# Autodesk Inventor assembly: Subensamble_cortadora_MIR
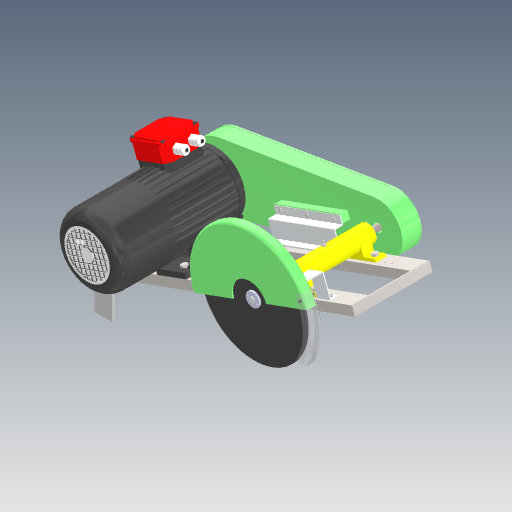
[picture p0: Inventor's stored thumbnail of the model, 512x512]
Saved by Autodesk Inventor 2021 (Build 250183000, 183)
## iProperties
Created: 2009-02-21
Part Number: Subensamble_cortadora_MIR
Document SubType Name: Assembly
Designer: maaro
Sending System: SolidWorks 2010
Last Author: Dominic
Last Saved: 2012-06-29
Author: Admin
## Documents named in this file (4)
- C:\Users\maaro\Documents\UNAL\Automatización de Procesos de Manufactura\Github\Proyecto_APM\CADs estaciones a automatizar\Estación corte\Subensamble_cortadora_MIR.iam
- C:\Users\maaro\Documents\UNAL\Automatización de Procesos de Manufactura\Github\Proyecto_APM\CADs estaciones a automatizar\Estación corte\belt cover lid_MIR.ipt
- C:\Users\maaro\Documents\UNAL\Automatización de Procesos de Manufactura\Github\Proyecto_APM\CADs estaciones a automatizar\Estación corte\Grupo_cortadora_MIR.iam
- C:\Users\maaro\Documents\UNAL\Automatización de Procesos de Manufactura\Github\Proyecto_APM\CADs estaciones a automatizar\Estación corte\Subensamble_Base cortadora_MIR.iam
## Components (3 placed, 3 different names)
1. belt cover lid_MIR:1 — Mate:1, Mate:2, Mate:3
2. Grupo_cortadora_MIR:1 [sub-assembly] — Rotational:1, Mate:1, Mate:2, Mate:3
3. Subensamble_Base cortadora_MIR:1 [sub-assembly] — Rotational:1
## Relationships (4: Mate 3, RevoluteJoint 1)
- Rotational:1 [RevoluteJoint] (0.05 mm): Grupo_cortadora_MIR:1 ↔ Subensamble_Base cortadora_MIR:1
- Mate:1: belt cover lid_MIR:1 ↔ Grupo_cortadora_MIR:1
- Mate:2: belt cover lid_MIR:1 ↔ Grupo_cortadora_MIR:1
- Mate:3: belt cover lid_MIR:1 ↔ Grupo_cortadora_MIR:1
